# Autodesk Inventor assembly: Ratchet System 1764
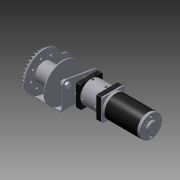
[picture p0: Inventor's stored thumbnail of the model, 180x180]
Saved by Autodesk Inventor 2011 (Build 150239000, 239)
## iProperties
Created: 2010-02-05
Part Number: Ratchet System 1764
Document SubType Name: Assembly
Designer: jrobinson
Author: jrobinson
## Documents named in this file (8)
- R:\CAD Archives\Manipulators\Ratchet System 1764 Needs Work\Ratchet System 1764.iam
- R:\CAD Archives\Manipulators\Ratchet System 1764 Needs Work\Ratchet Frame 1764.ipt
- R:\CAD Archives\Manipulators\Ratchet System 1764 Needs Work\Ratchet Bushing 1764.ipt
- R:\CAD Archives\Manipulators\Ratchet System 1764 Needs Work\Bolt 1764.ipt
- R:\CAD Archives\Manipulators\Ratchet System 1764 Needs Work\Big Nut 1764.ipt
- R:\CAD Archives\Manipulators\Ratchet System 1764 Needs Work\Spool 1764.ipt
- R:\CAD Archives\Manipulators\Ratchet System 1764 Needs Work\Bushing 1764.ipt
- R:\CAD Archives\Manipulators\Ratchet System 1764 Needs Work\Ratchet Sprocket Gears 1764.iam
## Components (9 placed, 8 different names)
1. Ratchet Frame 1764:1 — Mate:1, Mate:2, Mate:3, Mate:4, Angle:3, Mate:11, Angle:4, Mate:12, Mate:14, Mate:18, Mate:20, Angle:6
2. Ratchet Bushing 1764:1 — Mate:1, Mate:2, Mate:5
3. Ratchet Bushing 1764:2 — Mate:3, Mate:4, Mate:21, Mate:23
4. Ratchet Sprocket Gears 1764:1 [sub-assembly] — Mate:5, Angle:3, Mate:15, Angle:5, Mate:22
5. CIM Motor Bane Bots 1764:1 [sub-assembly] — Mate:21, Mate:22, Mate:23, Angle:6
6. Bolt 1764:1 — Mate:11, Angle:4, Mate:12, Mate:13, Mate:15, Mate:16
7. Big Nut 1764:1 — Mate:13, Mate:14
8. Spool 1764:1 — Mate:16, Mate:18, Angle:5, Mate:19
9. Bushing 1764:1 — Mate:19, Mate:20
## Relationships (21: Mate 17, Angle 4)
- Mate:1: Ratchet Frame 1764:1 ↔ Ratchet Bushing 1764:1
- Mate:2: Ratchet Frame 1764:1 ↔ Ratchet Bushing 1764:1
- Mate:3: Ratchet Frame 1764:1 ↔ Ratchet Bushing 1764:2
- Mate:4: Ratchet Frame 1764:1 ↔ Ratchet Bushing 1764:2
- Mate:5: Ratchet Bushing 1764:1 ↔ Ratchet Sprocket Gears 1764:1
- Angle:3 (0 deg): Ratchet Frame 1764:1 ↔ Ratchet Sprocket Gears 1764:1
- Mate:11: Ratchet Frame 1764:1 ↔ Bolt 1764:1
- Angle:4 (180 deg): Ratchet Frame 1764:1 ↔ Bolt 1764:1
- Mate:12: Ratchet Frame 1764:1 ↔ Bolt 1764:1
- Mate:13: Bolt 1764:1 ↔ Big Nut 1764:1
- Mate:14: Ratchet Frame 1764:1 ↔ Big Nut 1764:1
- Mate:15: Ratchet Sprocket Gears 1764:1 ↔ Bolt 1764:1
- Mate:16: Bolt 1764:1 ↔ Spool 1764:1
- Mate:18: Ratchet Frame 1764:1 ↔ Spool 1764:1
- Angle:5 (90 deg): Ratchet Sprocket Gears 1764:1 ↔ Spool 1764:1
- Mate:19: Spool 1764:1 ↔ Bushing 1764:1
- Mate:20: Ratchet Frame 1764:1 ↔ Bushing 1764:1
- Mate:21: Ratchet Bushing 1764:2 ↔ CIM Motor Bane Bots 1764:1
- Mate:22: Ratchet Sprocket Gears 1764:1 ↔ CIM Motor Bane Bots 1764:1
- Mate:23: Ratchet Bushing 1764:2 ↔ CIM Motor Bane Bots 1764:1
- Angle:6 (0 deg): Ratchet Frame 1764:1 ↔ CIM Motor Bane Bots 1764:1
